# Autodesk Inventor assembly: FootLeft
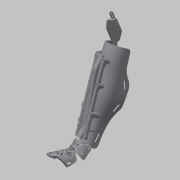
[picture p0: Inventor's stored thumbnail of the model, 180x180]
Saved by Autodesk Inventor 2015 SP1 (Build 190203100, 203)
## iProperties
Created: 2014-12-25
Part Number: FootLeft
Document SubType Name: Assembly
Designer: Val
Author: Val
## Documents named in this file (8)
- C:\Users\Val\Desktop\ExoGit\elysium-max-exoskeleton\src\Assemblies\LegRight.iam
- C:\Users\Val\Desktop\ExoGit\elysium-max-exoskeleton\src\FootShockPlate.ipt
- C:\Users\Val\Desktop\ExoGit\elysium-max-exoskeleton\src\FootUpperShockPlate.ipt
- C:\Users\Val\Desktop\ExoGit\elysium-max-exoskeleton\src\ShinShockPlateRight.ipt
- C:\Users\Val\Desktop\ExoGit\elysium-max-exoskeleton\src\ShinConnectorRight.ipt
- C:\Users\Val\Desktop\ExoGit\elysium-max-exoskeleton\src\ShinRight.ipt
- C:\Users\Val\Desktop\ExoGit\elysium-max-exoskeleton\src\ShinLockRight.ipt
- C:\Users\Val\Desktop\ExoGit\elysium-max-exoskeleton\src\ShinExtender.ipt
## Components (7 placed, 7 different names)
1. FootShockPlate:1
2. FootUpperShockPlate:1
3. ShinShockPlateRight:1 — Mate:1, Mate:2, Mate:3
4. ShinConnectorRight:1 — Mate:7, Mate:8, Mate:9, Mate:10, Mate:11, Mate:12
5. ShinRight:1 — Mate:1, Mate:2, Mate:3, Mate:4, Mate:5, Mate:6, Mate:8, Mate:9, Mate:10
6. ShinLockRight:1 — Mate:4, Mate:5, Mate:6
7. ShinExtender:1 — Mate:7, Mate:11, Mate:12
## Relationships (12: Mate 12)
- Mate:1: ShinShockPlateRight:1 ↔ ShinRight:1
- Mate:2: ShinShockPlateRight:1 ↔ ShinRight:1
- Mate:3: ShinShockPlateRight:1 ↔ ShinRight:1
- Mate:4: ShinRight:1 ↔ ShinLockRight:1
- Mate:5: ShinRight:1 ↔ ShinLockRight:1
- Mate:6: ShinRight:1 ↔ ShinLockRight:1
- Mate:7: ShinConnectorRight:1 ↔ ShinExtender:1
- Mate:8: ShinConnectorRight:1 ↔ ShinRight:1
- Mate:9: ShinConnectorRight:1 ↔ ShinRight:1
- Mate:10: ShinConnectorRight:1 ↔ ShinRight:1
- Mate:11: ShinConnectorRight:1 ↔ ShinExtender:1
- Mate:12: ShinConnectorRight:1 ↔ ShinExtender:1
